# Autodesk Inventor assembly: ASM0002_ASM
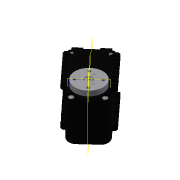
[picture p0: Inventor's stored thumbnail of the model, 180x180]
Saved by Autodesk Inventor 2016 (Build 200138000, 138)
## iProperties
Created: 2015-12-08
Part Number: ASM0002_ASM
Document SubType Name: Assembly
Designer: Bartłomiej Graca
Author: Bartłomiej Graca
## Documents named in this file (7)
- D:\PROJECTS\2016_biped\hermes\mechanics_tmp\ASM0002_ASM.iam
- D:\PROJECTS\2016_biped\hermes\mechanics_tmp\PRT0001.ipt
- D:\PROJECTS\2016_biped\hermes\mechanics_tmp\PRT0002.ipt
- D:\PROJECTS\2016_biped\hermes\mechanics_tmp\PRT0003.ipt
- D:\PROJECTS\2016_biped\hermes\mechanics_tmp\PRT0005.ipt
- D:\PROJECTS\2016_biped\hermes\mechanics_tmp\PRT0006.ipt
- D:\PROJECTS\2016_biped\hermes\mechanics_tmp\PRT0007.ipt
## Components (9 placed, 9 different names)
1. PRT0001_0 — Zestawiający:1, Mate:2, Mate:4, Zestawiający:7, Wstaw:1, Wstaw:2, Wstaw:3, Wstaw:4, Wstaw:5, Mate:8
2. PRT0002_1 — Zestawiający:1, Mate:2, Zestawiający:3, Mate:5
3. PRT0003_2 — Wstaw:3
4. PRT0003_3 — Wstaw:4
5. PRT0003_4 — Wstaw:5
6. PRT0003_5 — Wstaw:2
7. PRT0005_8 — Wstaw:1
8. PRT0006_9 — Zestawiający:3, Mate:4, Mate:5, Mate:6, Mate:8
9. PRT0007_10 — Mate:6, Zestawiający:7
## Relationships (13: Mate 8, Insert 5)
- Zestawiający:1 [Mate]: PRT0001_0 ↔ PRT0002_1
- Mate:2: PRT0001_0 ↔ PRT0002_1
- Zestawiający:3 [Mate]: PRT0002_1 ↔ PRT0006_9
- Mate:4: PRT0001_0 ↔ PRT0006_9
- Mate:5: PRT0002_1 ↔ PRT0006_9
- Mate:6: PRT0006_9 ↔ PRT0007_10
- Zestawiający:7 [Mate]: PRT0001_0 ↔ PRT0007_10
- Wstaw:1 [Insert]: PRT0001_0 ↔ PRT0005_8
- Wstaw:2 [Insert]: PRT0001_0 ↔ PRT0003_5
- Wstaw:3 [Insert]: PRT0001_0 ↔ PRT0003_2
- Wstaw:4 [Insert]: PRT0001_0 ↔ PRT0003_3
- Wstaw:5 [Insert]: PRT0001_0 ↔ PRT0003_4
- Mate:8: PRT0001_0 ↔ PRT0006_9
